# Autodesk Inventor assembly: Assembly2
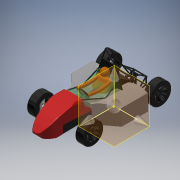
[picture p0: Inventor's stored thumbnail of the model, 180x180]
Saved by Autodesk Inventor 2018.1 (Build 221171000, 171)
## iProperties
Created: 2017-10-26
Part Number: Assembly2
Material: 一般
Document SubType Name: Assembly
Designer: KITformula
Author: KITformula
## Documents named in this file (4)
- C:\Users\formula\Dropbox\ishizaka\side1\Assembly2.iam
- D:\formula\ドキュメント\Inventor\ishizaka\KS-14_SLow\KS-14_SLow.iam
- C:\Users\formula\Dropbox\ishizaka\side1\part\ishispe.ipt
- C:\Users\formula\Dropbox\ishizaka\side1\part\ishispe_MIR.ipt
## Components (3 placed, 3 different names)
1. KS-14_SLow:1 [sub-assembly] — メイト:1, フラッシュ:1, 正接:1
2. ishispe:1 — フラッシュ:2, フラッシュ:3, フラッシュ:4
3. ishispe_MIR:1 — フラッシュ:5, メイト:2, メイト:3
## Relationships (9: Flush 5, Mate 3, Tangent 1)
- メイト:1 [Mate]: KS-14_SLow:1
- フラッシュ:1 [Flush]: KS-14_SLow:1
- 正接:1 [Tangent]: KS-14_SLow:1
- フラッシュ:2 [Flush]: ishispe:1
- フラッシュ:3 [Flush]: ishispe:1
- フラッシュ:4 [Flush]: ishispe:1
- フラッシュ:5 [Flush]: ishispe_MIR:1
- メイト:2 [Mate]: ishispe_MIR:1
- メイト:3 [Mate]: ishispe_MIR:1
